# Autodesk Inventor assembly: Casing
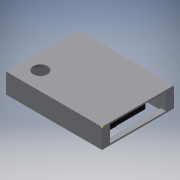
[picture p0: Inventor's stored thumbnail of the model, 180x180]
Saved by Autodesk Inventor 2017 (Build 210142000, 142)
## iProperties
Created: 2020-01-23
Part Number: Casing
Document SubType Name: Assembly
Designer: Manny
Author: Manny
## Documents named in this file (3)
- C:\Users\Owner\Documents\ENG Year 5\Casing.iam
- C:\Users\Owner\Documents\ENG Year 5\Rpi3Bplus.ipt
- C:\Users\Owner\Documents\ENG Year 5\Case_Top_Part.ipt
## Components (2 placed, 2 different names)
1. Rpi3Bplus:1 — Flush:1
2. Case_Top_Part:1 — Flush:1
## Relationships (1: Flush 1)
- Flush:1: Rpi3Bplus:1 ↔ Case_Top_Part:1
